# Autodesk Inventor assembly: Assem1
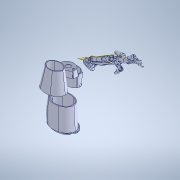
[picture p0: Inventor's stored thumbnail of the model, 180x180]
Saved by Autodesk Inventor 2022 (Build 260153000, 153)
## iProperties
Created: 2021-11-28
Part Number: Assem1
Document SubType Name: Assembly
Designer: User
Author: User
## Documents named in this file (37)
- D:\Users\Fer!\OneDrive - ESCUELA COLOMBIANA DE INGENIERIA JULIO GARAVITO\Escritorio\UNIVERSITY\roobotic_hand\robotic hand\aseembly\Assem1.iam
- D:\Users\Fer!\OneDrive - ESCUELA COLOMBIANA DE INGENIERIA JULIO GARAVITO\Escritorio\UNIVERSITY\roobotic_hand\robotic hand\aseembly\1.ipt
- D:\Users\Fer!\OneDrive - ESCUELA COLOMBIANA DE INGENIERIA JULIO GARAVITO\Escritorio\UNIVERSITY\roobotic_hand\robotic hand\aseembly\2.ipt
- D:\Users\Fer!\OneDrive - ESCUELA COLOMBIANA DE INGENIERIA JULIO GARAVITO\Escritorio\UNIVERSITY\roobotic_hand\robotic hand\aseembly\4.ipt
- D:\Users\Fer!\OneDrive - ESCUELA COLOMBIANA DE INGENIERIA JULIO GARAVITO\Escritorio\UNIVERSITY\roobotic_hand\robotic hand\aseembly\rotawrist1.ipt
- D:\Users\Fer!\OneDrive - ESCUELA COLOMBIANA DE INGENIERIA JULIO GARAVITO\Escritorio\UNIVERSITY\roobotic_hand\robotic hand\aseembly\rotawrist2.ipt
- D:\Users\Fer!\OneDrive - ESCUELA COLOMBIANA DE INGENIERIA JULIO GARAVITO\Escritorio\UNIVERSITY\roobotic_hand\robotic hand\aseembly\rotawrist3.ipt
- D:\Users\Fer!\OneDrive - ESCUELA COLOMBIANA DE INGENIERIA JULIO GARAVITO\Escritorio\UNIVERSITY\roobotic_hand\robotic hand\aseembly\largewrist.ipt
- D:\Users\Fer!\OneDrive - ESCUELA COLOMBIANA DE INGENIERIA JULIO GARAVITO\Escritorio\UNIVERSITY\roobotic_hand\robotic hand\aseembly\vis3.ipt
- D:\Users\Fer!\OneDrive - ESCUELA COLOMBIANA DE INGENIERIA JULIO GARAVITO\Escritorio\UNIVERSITY\roobotic_hand\robotic hand\aseembly\smallwrist1.ipt
- D:\Users\Fer!\OneDrive - ESCUELA COLOMBIANA DE INGENIERIA JULIO GARAVITO\Escritorio\UNIVERSITY\roobotic_hand\robotic hand\aseembly\smallwrist2.ipt
- D:\Users\Fer!\OneDrive - ESCUELA COLOMBIANA DE INGENIERIA JULIO GARAVITO\Escritorio\UNIVERSITY\roobotic_hand\robotic hand\aseembly\vis1.ipt
- D:\Users\Fer!\OneDrive - ESCUELA COLOMBIANA DE INGENIERIA JULIO GARAVITO\Escritorio\UNIVERSITY\roobotic_hand\robotic hand\aseembly\thump6.ipt
- D:\Users\Fer!\OneDrive - ESCUELA COLOMBIANA DE INGENIERIA JULIO GARAVITO\Escritorio\UNIVERSITY\roobotic_hand\robotic hand\aseembly\vis2.ipt
- D:\Users\Fer!\OneDrive - ESCUELA COLOMBIANA DE INGENIERIA JULIO GARAVITO\Escritorio\UNIVERSITY\roobotic_hand\robotic hand\aseembly\thump4.ipt
- D:\Users\Fer!\OneDrive - ESCUELA COLOMBIANA DE INGENIERIA JULIO GARAVITO\Escritorio\UNIVERSITY\roobotic_hand\robotic hand\aseembly\thump3.ipt
- D:\Users\Fer!\OneDrive - ESCUELA COLOMBIANA DE INGENIERIA JULIO GARAVITO\Escritorio\UNIVERSITY\roobotic_hand\robotic hand\aseembly\thump2.ipt
- D:\Users\Fer!\OneDrive - ESCUELA COLOMBIANA DE INGENIERIA JULIO GARAVITO\Escritorio\UNIVERSITY\roobotic_hand\robotic hand\aseembly\thump0.ipt
- D:\Users\Fer!\OneDrive - ESCUELA COLOMBIANA DE INGENIERIA JULIO GARAVITO\Escritorio\UNIVERSITY\roobotic_hand\robotic hand\aseembly\index4.ipt
- D:\Users\Fer!\OneDrive - ESCUELA COLOMBIANA DE INGENIERIA JULIO GARAVITO\Escritorio\UNIVERSITY\roobotic_hand\robotic hand\aseembly\index3.ipt
- D:\Users\Fer!\OneDrive - ESCUELA COLOMBIANA DE INGENIERIA JULIO GARAVITO\Escritorio\UNIVERSITY\roobotic_hand\robotic hand\aseembly\index5.ipt
- D:\Users\Fer!\OneDrive - ESCUELA COLOMBIANA DE INGENIERIA JULIO GARAVITO\Escritorio\UNIVERSITY\roobotic_hand\robotic hand\aseembly\index6.ipt
- D:\Users\Fer!\OneDrive - ESCUELA COLOMBIANA DE INGENIERIA JULIO GARAVITO\Escritorio\UNIVERSITY\roobotic_hand\robotic hand\aseembly\index2.ipt
- D:\Users\Fer!\OneDrive - ESCUELA COLOMBIANA DE INGENIERIA JULIO GARAVITO\Escritorio\UNIVERSITY\roobotic_hand\robotic hand\aseembly\index1.ipt
- D:\Users\Fer!\OneDrive - ESCUELA COLOMBIANA DE INGENIERIA JULIO GARAVITO\Escritorio\UNIVERSITY\roobotic_hand\robotic hand\aseembly\majeur4.ipt
- D:\Users\Fer!\OneDrive - ESCUELA COLOMBIANA DE INGENIERIA JULIO GARAVITO\Escritorio\UNIVERSITY\roobotic_hand\robotic hand\aseembly\majeur3.ipt
- D:\Users\Fer!\OneDrive - ESCUELA COLOMBIANA DE INGENIERIA JULIO GARAVITO\Escritorio\UNIVERSITY\roobotic_hand\robotic hand\aseembly\majeur5.ipt
- D:\Users\Fer!\OneDrive - ESCUELA COLOMBIANA DE INGENIERIA JULIO GARAVITO\Escritorio\UNIVERSITY\roobotic_hand\robotic hand\aseembly\majeur1.ipt
- D:\Users\Fer!\OneDrive - ESCUELA COLOMBIANA DE INGENIERIA JULIO GARAVITO\Escritorio\UNIVERSITY\roobotic_hand\robotic hand\aseembly\majeur2.ipt
- D:\Users\Fer!\OneDrive - ESCUELA COLOMBIANA DE INGENIERIA JULIO GARAVITO\Escritorio\UNIVERSITY\roobotic_hand\robotic hand\aseembly\majeur6.ipt
- D:\Users\Fer!\OneDrive - ESCUELA COLOMBIANA DE INGENIERIA JULIO GARAVITO\Escritorio\UNIVERSITY\roobotic_hand\robotic hand\aseembly\auriculaire4.ipt
- D:\Users\Fer!\OneDrive - ESCUELA COLOMBIANA DE INGENIERIA JULIO GARAVITO\Escritorio\UNIVERSITY\roobotic_hand\robotic hand\aseembly\auriculaire3.ipt
- D:\Users\Fer!\OneDrive - ESCUELA COLOMBIANA DE INGENIERIA JULIO GARAVITO\Escritorio\UNIVERSITY\roobotic_hand\robotic hand\aseembly\auriculaire1.ipt
- D:\Users\Fer!\OneDrive - ESCUELA COLOMBIANA DE INGENIERIA JULIO GARAVITO\Escritorio\UNIVERSITY\roobotic_hand\robotic hand\aseembly\auriculaire2.ipt
- D:\Users\Fer!\OneDrive - ESCUELA COLOMBIANA DE INGENIERIA JULIO GARAVITO\Escritorio\UNIVERSITY\roobotic_hand\robotic hand\aseembly\auriculaire5.ipt
- D:\Users\Fer!\OneDrive - ESCUELA COLOMBIANA DE INGENIERIA JULIO GARAVITO\Escritorio\UNIVERSITY\roobotic_hand\robotic hand\aseembly\auriculaire6.ipt
- D:\Users\Fer!\OneDrive - ESCUELA COLOMBIANA DE INGENIERIA JULIO GARAVITO\Escritorio\UNIVERSITY\roobotic_hand\robotic hand\My assembly\thump5.ipt
## Components (42 placed, 36 different names)
1. 1:1
2. 2:1
3. 4:1
4. rotawrist1:1
5. rotawrist2:1
6. rotawrist3:1 — Coincidencia:68, Coincidencia:69
7. largewrist:1 — Ángulo:2, Tangente:1, Ángulo:3, Insertar:1, Insertar:2, Insertar:3, Coincidencia:12, Coincidencia:13, Coincidencia:14, Coincidencia:15, Coincidencia:16, Coincidencia:17, Coincidencia:51, Coincidencia:53, Coincidencia:64, Coincidencia:65, Coincidencia:69
8. vis3:1 — Insertar:2, Coincidencia:68
9. smallwrist1:1 — Coincidencia:15, Coincidencia:16, Coincidencia:40, Coincidencia:41
10. smallwrist2:1 — Coincidencia:14, Coincidencia:17, Coincidencia:27, Coincidencia:28
11. vis1:1 — Insertar:1
12. thump6:1 — Coincidencia:7, Coincidencia:10, Coincidencia:11, Coincidencia:12, Coincidencia:13
13. vis2:1 — Insertar:3
14. thump4:1 — Coincidencia:5, Coincidencia:6, Coincidencia:8, Coincidencia:9, Ángulo:1
15. thump3:1 — Coincidencia:3, Coincidencia:4, Coincidencia:8, Coincidencia:9, Ángulo:1
16. thump2:1 — Coincidencia:1, Coincidencia:2, Coincidencia:3, Coincidencia:4
17. thump0:1 — Coincidencia:1, Coincidencia:2
18. index4:1 — Coincidencia:62, Coincidencia:63, Coincidencia:64, Coincidencia:65
19. index3:1 — Coincidencia:60, Coincidencia:61, Coincidencia:62, Coincidencia:63
20. index5:1 — Coincidencia:58, Coincidencia:59, Coincidencia:60, Coincidencia:61
21. index6:1 — Coincidencia:56, Coincidencia:57, Coincidencia:58, Coincidencia:59
22. index2:1 — Coincidencia:54, Coincidencia:55, Coincidencia:56, Coincidencia:57
23. index1:1 — Coincidencia:54, Coincidencia:55
24. majeur4:1 — Coincidencia:50, Coincidencia:51, Coincidencia:52, Coincidencia:53
25. majeur3:1 — Coincidencia:48, Coincidencia:49, Coincidencia:50, Coincidencia:52
26. majeur5:1 — Coincidencia:46, Coincidencia:47, Coincidencia:48, Coincidencia:49
27. majeur1:1 — Coincidencia:42, Coincidencia:43
28. majeur2:1 — Coincidencia:42, Coincidencia:43, Coincidencia:44, Coincidencia:45
29. majeur6:1 — Coincidencia:44, Coincidencia:45, Coincidencia:46, Coincidencia:47
30. index3:2 — Coincidencia:36, Coincidencia:37, Coincidencia:38, Coincidencia:39, Ángulo:7, Ángulo:8
31. index4:2 — Coincidencia:38, Coincidencia:39, Coincidencia:40, Coincidencia:41, Ángulo:8
32. index1:2 — Coincidencia:30, Coincidencia:31, Coincidencia:70
33. index2:2 — Coincidencia:30, Coincidencia:31, Coincidencia:32, Coincidencia:33, Coincidencia:70
34. index5:2 — Coincidencia:34, Coincidencia:35, Coincidencia:36, Coincidencia:37
35. index6:2 — Coincidencia:32, Coincidencia:33, Coincidencia:34, Coincidencia:35, Ángulo:7
36. auriculaire4:2 — Coincidencia:26, Coincidencia:27, Coincidencia:28, Coincidencia:29, Ángulo:6
37. auriculaire3:1 — Coincidencia:24, Coincidencia:25, Coincidencia:26, Coincidencia:29, Ángulo:6
38. auriculaire1:1 — Coincidencia:18, Coincidencia:19
39. auriculaire2:1 — Coincidencia:18, Coincidencia:19, Coincidencia:20, Coincidencia:21
40. auriculaire5:1 — Coincidencia:22, Coincidencia:23, Coincidencia:24, Coincidencia:25, Ángulo:5
41. auriculaire6:1 — Coincidencia:20, Coincidencia:21, Coincidencia:22, Coincidencia:23, Ángulo:5
42. thump5:1 — Coincidencia:5, Coincidencia:6, Coincidencia:7, Coincidencia:10, Coincidencia:11
## Relationships (79: Mate 68, Angle 7, Insert 3, Tangent 1)
- Coincidencia:1 [Mate]: thump2:1 ↔ thump0:1
- Coincidencia:2 [Mate]: thump2:1 ↔ thump0:1
- Coincidencia:3 [Mate]: thump3:1 ↔ thump2:1
- Coincidencia:4 [Mate]: thump3:1 ↔ thump2:1
- Coincidencia:5 [Mate]: thump4:1 ↔ thump5:1
- Coincidencia:6 [Mate]: thump4:1 ↔ thump5:1
- Coincidencia:7 [Mate]: thump6:1 ↔ thump5:1
- Coincidencia:8 [Mate]: thump4:1 ↔ thump3:1
- Coincidencia:9 [Mate]: thump4:1 ↔ thump3:1
- Ángulo:1 [Angle] (180 deg): thump4:1 ↔ thump3:1
- Coincidencia:10 [Mate]: thump6:1 ↔ thump5:1
- Coincidencia:11 [Mate]: thump6:1 ↔ thump5:1
- Ángulo:2 [Angle] (0 deg): largewrist:1
- Tangente:1: largewrist:1
- Ángulo:3 [Angle] (0 deg): largewrist:1
- Insertar:1: largewrist:1 ↔ vis1:1
- Insertar:2: largewrist:1 ↔ vis3:1
- Insertar:3: largewrist:1 ↔ vis2:1
- Coincidencia:12 [Mate]: largewrist:1 ↔ thump6:1
- Coincidencia:13 [Mate]: largewrist:1 ↔ thump6:1
- Coincidencia:14 [Mate]: largewrist:1 ↔ smallwrist2:1
- Coincidencia:15 [Mate]: largewrist:1 ↔ smallwrist1:1
- Coincidencia:16 [Mate]: largewrist:1 ↔ smallwrist1:1
- Coincidencia:17 [Mate] (0.5 mm): largewrist:1 ↔ smallwrist2:1
- Coincidencia:18 [Mate]: auriculaire1:1 ↔ auriculaire2:1
- Coincidencia:19 [Mate]: auriculaire1:1 ↔ auriculaire2:1
- Coincidencia:20 [Mate]: auriculaire2:1 ↔ auriculaire6:1
- Coincidencia:21 [Mate]: auriculaire2:1 ↔ auriculaire6:1
- Coincidencia:22 [Mate]: auriculaire5:1 ↔ auriculaire6:1
- Coincidencia:23 [Mate]: auriculaire5:1 ↔ auriculaire6:1
- Coincidencia:24 [Mate]: auriculaire3:1 ↔ auriculaire5:1
- Coincidencia:25 [Mate]: auriculaire3:1 ↔ auriculaire5:1
- Coincidencia:26 [Mate]: auriculaire4:2 ↔ auriculaire3:1
- Coincidencia:27 [Mate]: smallwrist2:1 ↔ auriculaire4:2
- Coincidencia:28 [Mate]: smallwrist2:1 ↔ auriculaire4:2
- Coincidencia:29 [Mate]: auriculaire4:2 ↔ auriculaire3:1
- Coincidencia:30 [Mate]: index1:2 ↔ index2:2
- Coincidencia:31 [Mate]: index1:2 ↔ index2:2
- Coincidencia:32 [Mate]: index2:2 ↔ index6:2
- Coincidencia:33 [Mate]: index2:2 ↔ index6:2
- Coincidencia:34 [Mate]: index5:2 ↔ index6:2
- Coincidencia:35 [Mate]: index5:2 ↔ index6:2
- Coincidencia:36 [Mate]: index3:2 ↔ index5:2
- Coincidencia:37 [Mate]: index3:2 ↔ index5:2
- Coincidencia:38 [Mate]: index3:2 ↔ index4:2
- Coincidencia:39 [Mate]: index3:2 ↔ index4:2
- Coincidencia:40 [Mate]: smallwrist1:1 ↔ index4:2
- Coincidencia:41 [Mate]: smallwrist1:1 ↔ index4:2
- Coincidencia:42 [Mate]: majeur1:1 ↔ majeur2:1
- Coincidencia:43 [Mate]: majeur1:1 ↔ majeur2:1
- Coincidencia:44 [Mate]: majeur2:1 ↔ majeur6:1
- Coincidencia:45 [Mate]: majeur2:1 ↔ majeur6:1
- Coincidencia:46 [Mate]: majeur5:1 ↔ majeur6:1
- Coincidencia:47 [Mate]: majeur5:1 ↔ majeur6:1
- Coincidencia:48 [Mate]: majeur3:1 ↔ majeur5:1
- Coincidencia:49 [Mate]: majeur3:1 ↔ majeur5:1
- Coincidencia:50 [Mate]: majeur4:1 ↔ majeur3:1
- Coincidencia:51 [Mate]: largewrist:1 ↔ majeur4:1
- Coincidencia:52 [Mate]: majeur4:1 ↔ majeur3:1
- Coincidencia:53 [Mate]: largewrist:1 ↔ majeur4:1
- Coincidencia:54 [Mate]: index2:1 ↔ index1:1
- Coincidencia:55 [Mate]: index2:1 ↔ index1:1
- Coincidencia:56 [Mate]: index6:1 ↔ index2:1
- Coincidencia:57 [Mate]: index6:1 ↔ index2:1
- Coincidencia:58 [Mate]: index5:1 ↔ index6:1
- Coincidencia:59 [Mate]: index5:1 ↔ index6:1
- Coincidencia:60 [Mate]: index3:1 ↔ index5:1
- Coincidencia:61 [Mate]: index3:1 ↔ index5:1
- Coincidencia:62 [Mate]: index4:1 ↔ index3:1
- Coincidencia:63 [Mate]: index4:1 ↔ index3:1
- Coincidencia:64 [Mate]: largewrist:1 ↔ index4:1
- Coincidencia:65 [Mate]: largewrist:1 ↔ index4:1
- Coincidencia:68 [Mate]: rotawrist3:1 ↔ vis3:1
- Coincidencia:69 [Mate]: rotawrist3:1 ↔ largewrist:1
- Ángulo:5 [Angle] (180 deg): auriculaire5:1 ↔ auriculaire6:1
- Ángulo:6 [Angle] (180 deg): auriculaire4:2 ↔ auriculaire3:1
- Ángulo:7 [Angle] (0 deg): index3:2 ↔ index6:2
- Ángulo:8 [Angle] (180 deg): index3:2 ↔ index4:2
- Coincidencia:70 [Mate]: index1:2 ↔ index2:2
